# Autodesk Inventor assembly: CL-6-F
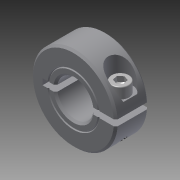
[picture p0: Inventor's stored thumbnail of the model, 180x180]
Saved by Autodesk Inventor 2013 (Build 170138000, 138)
## iProperties
Category: Miscellaneous
Company: Autodesk Inc.
Created: 2012-12-03
Part Number: CL-6-F
Document SubType Name: Assembly
Designer: Autodesk Inc.
Catalog Web Link: http://www.ruland.com/ps_collars_shaft_cl.asp
Description: 3/8" ID 7/8" OD Clamp Shaft Collar
Vendor: Ruland Manufacturing
Author: Autodesk Inc.
## Documents named in this file (3)
- C:\Data Folder\FIRST 2013\FIRST KOP\Parts\Miscellaneous\MISC_ShaftCollar_CL-6-F.iam
- C:\Data Folder\FIRST 2013\FIRST KOP\Parts\Miscellaneous\MISC_ShaftCollar_CL-6-F.ipt
- C:\Data Folder\FIRST 2013\FIRST KOP\Parts\Miscellaneous\ANSI B18.3 - 4-40 UNC - 0.25(31).ipt
## Components (2 placed, 2 different names)
1. MISC_ShaftCollar_CL-6-F:1 — Mate:1, Insert:1
2. Hexagon Socket Head Cap Screw - Inch No. 4 - 40 UNC - 1/4:1 — Mate:1, Insert:1
## Relationships (2: Insert 1, Mate 1)
- Insert:1: MISC_ShaftCollar_CL-6-F:1 ↔ Hexagon Socket Head Cap Screw - Inch No. 4 - 40 UNC - 1/4:1
- Mate:1: MISC_ShaftCollar_CL-6-F:1 ↔ Hexagon Socket Head Cap Screw - Inch No. 4 - 40 UNC - 1/4:1
